# Autodesk Inventor assembly: mg996r 3mm legs
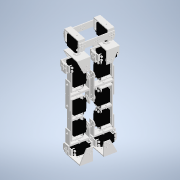
[picture p0: Inventor's stored thumbnail of the model, 180x180]
Saved by Autodesk Inventor 2021.4 (Build 254397000, 397)
## iProperties
Created: 2022-07-09
Part Number: mg996r 3mm legs
Document SubType Name: Assembly
Designer: isamu
Author: isamu
## Documents named in this file (5)
- D:\personal_projects\robot\inventor\2021\mg996r 3mm legs.iam
- D:\personal_projects\robot\inventor\2021\mg996 3mm top.iam
- D:\personal_projects\robot\inventor\2021\mg996r 3mm left leg.iam
- D:\personal_projects\robot\inventor\2021\mg996r 3mm right leg.iam
- D:\personal_projects\robot\exports\screws\m2 nuts.ipt
## Components (11 placed, 4 different names)
1. mg996 3mm top:1 [sub-assembly] — Mate:1, Mate:2, Mate:3, Mate:4, Mate:5, Mate:6
2. mg996r 3mm left leg:1 [sub-assembly] — Insert:5, Insert:6, Insert:7, Insert:8, Mate:1, Mate:2, Mate:3
3. mg996r 3mm right leg:1 [sub-assembly] — Insert:1, Insert:2, Insert:3, Insert:4, Mate:4, Mate:5, Mate:6
4. m2 nuts:1 — Insert:2
5. m2 nuts:2 — Insert:4
6. m2 nuts:3 — Insert:6
7. m2 nuts:4 — Insert:1
8. m2 nuts:5 — Insert:5
9. m2 nuts:6 — Insert:8
10. m2 nuts:7 — Insert:7
11. m2 nuts:8 — Insert:3
## Relationships (14: Insert 8, Mate 6)
- Insert:1: mg996r 3mm right leg:1 ↔ m2 nuts:4
- Insert:2: mg996r 3mm right leg:1 ↔ m2 nuts:1
- Insert:3: mg996r 3mm right leg:1 ↔ m2 nuts:8
- Insert:4: mg996r 3mm right leg:1 ↔ m2 nuts:2
- Insert:5: mg996r 3mm left leg:1 ↔ m2 nuts:5
- Insert:6: mg996r 3mm left leg:1 ↔ m2 nuts:3
- Insert:7: mg996r 3mm left leg:1 ↔ m2 nuts:7
- Insert:8: mg996r 3mm left leg:1 ↔ m2 nuts:6
- Mate:1: mg996 3mm top:1 ↔ mg996r 3mm left leg:1
- Mate:2: mg996 3mm top:1 ↔ mg996r 3mm left leg:1
- Mate:3: mg996 3mm top:1 ↔ mg996r 3mm left leg:1
- Mate:4: mg996 3mm top:1 ↔ mg996r 3mm right leg:1
- Mate:5: mg996 3mm top:1 ↔ mg996r 3mm right leg:1
- Mate:6: mg996 3mm top:1 ↔ mg996r 3mm right leg:1
